# Autodesk Inventor assembly: Other Valve 1764
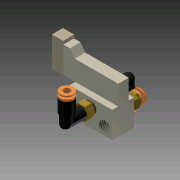
[picture p0: Inventor's stored thumbnail of the model, 180x180]
Saved by Autodesk Inventor 2011 (Build 150239000, 239)
## iProperties
Created: 2010-02-15
Part Number: Other Valve 1764
Document SubType Name: Assembly
Designer: jgehrig
Author: jgehrig
## Documents named in this file (5)
- R:\CAD Archives\Pnewmatics\Valve\Other Valve 1764.iam
- R:\CAD Archives\Pnewmatics\Valve\Valve Base 1764.ipt
- R:\CAD Archives\Pnewmatics\Valve\Valve Part 1764.ipt
- R:\CAD Archives\Pnewmatics\Pnematics Bend Piece\Bend Piece 1764.iam
- R:\CAD Archives\Pnewmatics\pnewmatic screw\Pnematic Screw 1764.iam
## Components (5 placed, 4 different names)
1. Valve Base 1764:1 — Flush:1, Mate:1, Flush:2, Insert:1, Insert:2, Angle:2, Insert:3
2. Valve Part 1764:1 — Flush:1, Mate:1, Flush:2, Angle:1
3. Bend Piece 1764:1 [sub-assembly] — Insert:1, Angle:1
4. Bend Piece 1764:2 [sub-assembly] — Insert:2, Angle:2
5. Pnematic Screw 1764:1 [sub-assembly] — Insert:3
## Relationships (8: Insert 3, Flush 2, Angle 2, Mate 1)
- Flush:1: Valve Base 1764:1 ↔ Valve Part 1764:1
- Mate:1: Valve Base 1764:1 ↔ Valve Part 1764:1
- Flush:2 (5.715 mm): Valve Base 1764:1 ↔ Valve Part 1764:1
- Insert:1: Valve Base 1764:1 ↔ Bend Piece 1764:1
- Angle:1 (0 deg): Valve Part 1764:1 ↔ Bend Piece 1764:1
- Insert:2: Valve Base 1764:1 ↔ Bend Piece 1764:2
- Angle:2 (0 deg): Valve Base 1764:1 ↔ Bend Piece 1764:2
- Insert:3: Valve Base 1764:1 ↔ Pnematic Screw 1764:1
